# Autodesk Inventor assembly: Complete7Segment
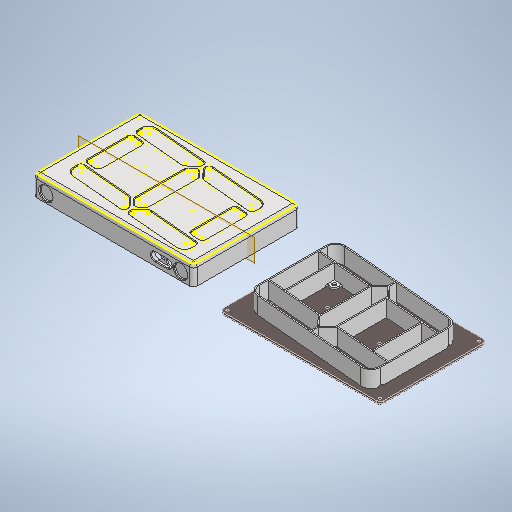
[picture p0: Inventor's stored thumbnail of the model, 512x512]
Saved by Autodesk Inventor 2025.2 (Build 292293000, 293)
## iProperties
Created: 2026-02-06
Part Number: Complete7Segment
Document SubType Name: Assembly
Designer: Joefi
Author: Joefi
## Documents named in this file (5)
- C:\Users\Joefi\source\repos\Seg7\Seg7_Hardware\Complete7Segment.iam
- C:\Users\Joefi\source\repos\Seg7\Seg7_Hardware\7Segment.ipt
- C:\Users\Joefi\source\repos\Seg7\Seg7_Hardware\BackPlate.ipt
- C:\Users\Joefi\source\repos\Seg7\Seg7_Hardware\Divider.ipt
- C:\Users\Joefi\source\repos\Seg7\Seg7_Hardware\SegmentPanels.ipt
## Components (5 placed, 4 different names)
1. 7Segment:1 — Mate:1, Mate:2, Flush:1, Flush:2, Mate:4
2. BackPlate:1 — Mate:1, Mate:2, Mate:3, Mate:4
3. Divider:1 — Flush:1, Flush:2, Mate:3
4. 7Segment:2 — Mate:5, Mate:6
5. SegmentPanels:1 — Mate:5, Mate:6
## Relationships (8: Mate 6, Flush 2)
- Mate:1: 7Segment:1 ↔ BackPlate:1
- Mate:2: 7Segment:1 ↔ BackPlate:1
- Flush:1: 7Segment:1 ↔ Divider:1
- Flush:2: 7Segment:1 ↔ Divider:1
- Mate:3: BackPlate:1 ↔ Divider:1
- Mate:4: 7Segment:1 ↔ BackPlate:1
- Mate:5: 7Segment:2 ↔ SegmentPanels:1
- Mate:6 (0.2 mm): 7Segment:2 ↔ SegmentPanels:1
